# Autodesk Inventor assembly: koks
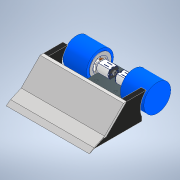
[picture p0: Inventor's stored thumbnail of the model, 180x180]
Saved by Autodesk Inventor 2022 (Build 260153000, 153)
## iProperties
Created: 2022-12-08
Part Number: koks
Document SubType Name: Assembly
Designer: Kamil
Author: Kamil
## Documents named in this file (8)
- C:\MiniSumo koks\koks.iam
- C:\MiniSumo koks\opona.ipt
- C:\MiniSumo koks\felga.ipt
- C:\MiniSumo koks\dół.ipt
- C:\MiniSumo koks\n20 motor.ipt
- C:\MiniSumo koks\podpora silników.ipt
- C:\MiniSumo koks\Part14.ipt
- C:\MiniSumo koks\nóż.ipt
## Components (10 placed, 7 different names)
1. felga:1 — Mate:5, Mate:6, Flush:5, Mate:9
2. felga:2 — Mate:7, Mate:8, Flush:4, Flush:6, Mate:10
3. dół:1 — Mate:1, Flush:1, Flush:2, Flush:4, Mate:11, Flush:7, Flush:8, Flush:10
4. n20 motor:1 — Mate:2, Flush:3, Mate:4, Mate:5, Mate:6
5. n20 motor:2 — Mate:2, Flush:3, Mate:3, Mate:4, Mate:7, Mate:8
6. podpora silników:1 — Mate:1, Flush:1, Flush:2, Mate:3
7. opona:1 — Flush:5, Mate:9, Mate:11
8. opona:2 — Flush:6, Mate:10
9. Part14:1 — Flush:7
10. nóż:1 — Flush:8, Flush:10
## Relationships (20: Mate 11, Flush 9)
- Mate:1: dół:1 ↔ podpora silników:1
- Flush:1: dół:1 ↔ podpora silników:1
- Flush:2: dół:1 ↔ podpora silników:1
- Mate:2 (5 mm): n20 motor:1 ↔ n20 motor:2
- Flush:3: n20 motor:1 ↔ n20 motor:2
- Mate:3: n20 motor:2 ↔ podpora silników:1
- Mate:4: n20 motor:1 ↔ n20 motor:2
- Mate:5: felga:1 ↔ n20 motor:1
- Mate:6 (0.5 mm): felga:1 ↔ n20 motor:1
- Mate:7: felga:2 ↔ n20 motor:2
- Mate:8 (0.5 mm): felga:2 ↔ n20 motor:2
- Flush:4 (-4.5 mm): felga:2 ↔ dół:1
- Flush:5 (-0.6 mm): felga:1 ↔ opona:1
- Mate:9: felga:1 ↔ opona:1
- Flush:6 (0.6 mm): felga:2 ↔ opona:2
- Mate:10: felga:2 ↔ opona:2
- Mate:11 (20.1 mm): dół:1 ↔ opona:1
- Flush:7: dół:1 ↔ Part14:1
- Flush:8: dół:1 ↔ nóż:1
- Flush:10: dół:1 ↔ nóż:1
